# Autodesk Inventor assembly: Manipulator
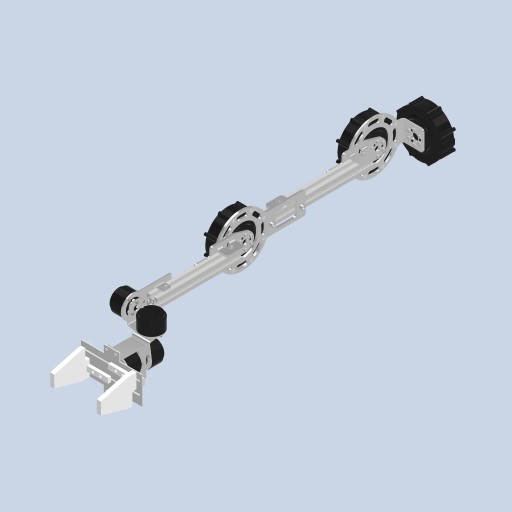
[picture p0: Inventor's stored thumbnail of the model, 512x512]
Saved by Autodesk Inventor 2023 (Build 270158000, 158)
## iProperties
Created: 2024-11-08
Part Number: Manipulator
Document SubType Name: Assembly
Designer: kiyo
Mass: 3708.17 g
Surface Area: 3992.73 cm^2
Volume: 794.407 cm^3
Density: 4.66785 g/cm^3
Author: kiyo
## Documents named in this file (20)
- D:\GitHub\inventor\syu-si\OfficeRobot\Manipulator\Manipulator.iam
- D:\GitHub\inventor\syu-si\OfficeRobot\ReadyMade\Steadywin\GIM8108-8.iam
- D:\GitHub\inventor\syu-si\OfficeRobot\ReadyMade\Steadywin\GIM3505-8_with-driver.ipt
- D:\GitHub\inventor\syu-si\OfficeRobot\Manipulator\wrist-pitch-plate.ipt
- D:\GitHub\inventor\syu-si\OfficeRobot\ReadyMade\Screw\FWSJJ-D5-V2_6-T4_5.ipt
- D:\GitHub\inventor\syu-si\OfficeRobot\ReadyMade\Screw\HNTU5-5.ipt
- D:\GitHub\inventor\syu-si\OfficeRobot\Manipulator\sholder_roll_bracket.ipt
- D:\GitHub\inventor\syu-si\OfficeRobot\ReadyMade\Screw\SCB5-8.ipt
- D:\GitHub\inventor\syu-si\OfficeRobot\ReadyMade\Aluminum-frame\NFS5-2020-170-AV15-BV145.ipt
- D:\GitHub\inventor\syu-si\OfficeRobot\Manipulator\wrist_bracket.ipt
- D:\GitHub\inventor\syu-si\OfficeRobot\Hand\Hand.iam
- D:\GitHub\inventor\syu-si\OfficeRobot\Manipulator\pitch_plate.ipt
- D:\GitHub\inventor\syu-si\OfficeRobot\ReadyMade\Screw\SCB5-25.ipt
- D:\GitHub\inventor\syu-si\OfficeRobot\ReadyMade\Screw\SCB5-10.ipt
- D:\GitHub\inventor\syu-si\OfficeRobot\Manipulator\elbow-pitch-plate_T4.ipt
- D:\GitHub\inventor\syu-si\OfficeRobot\ReadyMade\Screw\HFBCM3-8.ipt
- D:\GitHub\inventor\syu-si\OfficeRobot\ReadyMade\Aluminum-frame\NFS5-2020-215-AV15-BV180.ipt
- D:\GitHub\inventor\syu-si\OfficeRobot\ReadyMade\Screw\CBE3-8.ipt
- D:\GitHub\inventor\syu-si\OfficeRobot\ReadyMade\Screw\CSH-316L-M2_5-6.ipt
- D:\GitHub\inventor\syu-si\OfficeRobot\ReadyMade\Screw\CSH-316L-M2_5-10.ipt
## Components (101 placed, 19 different names)
1. sholder_roll_bracket:1 — 挿入:350, 挿入:414, 挿入:493, 挿入:517, 挿入:526, 挿入:527, 挿入:528, 挿入:529, 挿入:530, 挿入:531, 挿入:532, 挿入:533, 挿入:555, 挿入:556, 挿入:557, 挿入:558, 挿入:559, 挿入:573
2. pitch_plate:1 — 挿入:512, 正接:78, 正接:79, 正接:80, 角度:96, 挿入:561, 挿入:562, 挿入:563, 挿入:564, 挿入:565, 挿入:566
3. elbow-pitch-plate_T4:1 — 挿入:514, 挿入:515, 正接:83, 挿入:518, 挿入:519, 挿入:520, 挿入:521, 挿入:522, 挿入:523, 挿入:524, 挿入:525, 正接:84, 正接:85
4. pitch_plate:2 — 挿入:513, メイト:114, メイト:115, 正接:77, 正接:81, 正接:82, 角度:97, 挿入:567, 挿入:568, 挿入:569, 挿入:570, 挿入:571, 挿入:572, 正接:86
5. wrist-pitch-plate:1 — メイト:71, メイト:72, 正接:48, 正接:49, 角度:76, 角度:77, 角度:78, 正接:50, 正接:51, 挿入:470, 挿入:471
6. wrist_bracket:1
7. wrist_bracket:2 — 挿入:485
8. NFS5-2020-215-AV15-BV180:1
9. NFS5-2020-170-AV15-BV145:1 — メイト:106, メイト:107, 角度:90, 角度:91, 正接:70, 正接:71, 角度:92, メイト:108, 正接:74, 正接:75, メイト:114, メイト:115
10. Hand:1 [sub-assembly] — 挿入:497, 角度:98, 角度:99
11. CSH-316L-M2_5-6:1
12. CSH-316L-M2_5-6:2
13. CSH-316L-M2_5-6:3
14. CSH-316L-M2_5-6:4
15. CSH-316L-M2_5-6:5
16. CSH-316L-M2_5-6:6
17. CSH-316L-M2_5-6:7
18. CSH-316L-M2_5-6:8
19. CSH-316L-M2_5-6:9
20. CSH-316L-M2_5-10:1
21. CSH-316L-M2_5-10:2
22. CSH-316L-M2_5-10:3
23. CSH-316L-M2_5-10:4
24. CSH-316L-M2_5-10:5
25. CSH-316L-M2_5-10:6
26. CSH-316L-M2_5-10:7
27. CSH-316L-M2_5-10:8
28. CSH-316L-M2_5-10:9
29. CBE3-8:1 — 挿入:555
30. CBE3-8:2 — 挿入:557
31. CBE3-8:3 — 挿入:558
32. CBE3-8:4 — 挿入:573
33. CBE3-8:5 — 挿入:556
34. CBE3-8:6 — 挿入:559
35. CBE3-8:7 — 挿入:562
36. CBE3-8:8 — 挿入:561
37. CBE3-8:9 — 挿入:569
38. CBE3-8:10 — 挿入:572
39. CBE3-8:11 — 挿入:568
40. CBE3-8:12 — 挿入:563
41. CBE3-8:13 — 挿入:566
42. CBE3-8:14 — 挿入:567
43. CBE3-8:15 — 挿入:570
44. CBE3-8:16 — 挿入:571
45. CBE3-8:17 — 挿入:565
46. CBE3-8:18 — 挿入:564
47. HFBCM3-8:1 — 挿入:521
48. HFBCM3-8:2 — 挿入:524
49. HFBCM3-8:3 — 挿入:525
50. HFBCM3-8:4 — 挿入:523
51. HFBCM3-8:5 — 挿入:522
52. HFBCM3-8:6 — 挿入:518
53. HFBCM3-8:7 — 挿入:519
54. HFBCM3-8:8 — 挿入:520
55. HFBCM3-8:9 — 挿入:531
56. HFBCM3-8:10 — 挿入:532
57. HFBCM3-8:11 — 挿入:530
58. HFBCM3-8:12 — 挿入:529
59. HFBCM3-8:13 — 挿入:528
60. HFBCM3-8:14 — 挿入:533
61. HFBCM3-8:15 — 挿入:526
62. HFBCM3-8:16 — 挿入:527
63. FWSJJ-D5-V2_6-T4_5:16
64. FWSJJ-D5-V2_6-T4_5:17
65. FWSJJ-D5-V2_6-T4_5:18
66. FWSJJ-D5-V2_6-T4_5:10
67. FWSJJ-D5-V2_6-T4_5:11
68. FWSJJ-D5-V2_6-T4_5:12
69. FWSJJ-D5-V2_6-T4_5:13
70. FWSJJ-D5-V2_6-T4_5:14
71. FWSJJ-D5-V2_6-T4_5:15
72. SCB5-25:1 — 正接:78
73. SCB5-25:2 — メイト:108, 正接:74, 正接:75, 正接:77
74. SCB5-25:3 — 挿入:516, 正接:83
75. SCB5-25:4
76. SCB5-10:1 — 正接:80
77. SCB5-10:2 — 正接:79
78. SCB5-10:3 — メイト:106, 正接:70, 正接:82
79. SCB5-10:4 — メイト:107, 正接:71, 正接:81
80. SCB5-10:5 — 正接:85
81. SCB5-10:6 — 正接:84, 正接:86
82. SCB5-8:1 — 挿入:412, メイト:72, 正接:49, 正接:50
83. SCB5-8:2 — 挿入:411, メイト:71, 正接:48, 正接:51
84. HNTU5-5:1 — 角度:78
85. HNTU5-5:2 — 挿入:412, 角度:76
86. HNTU5-5:3 — 挿入:411, 角度:77
87. HNTU5-5:4 — 挿入:516
88. HNTU5-5:5
89. HNTU5-5:6
90. HNTU5-5:7
91. HNTU5-5:8 — 角度:90
92. HNTU5-5:9 — 角度:91
93. HNTU5-5:10 — 角度:92
94. HNTU5-5:11
95. HNTU5-5:12
96. GIM8108-8:1 [sub-assembly] — 挿入:350, 肩ピッチとの角度関係, 環境固定, 環境固定2
97. GIM8108-8:2 [sub-assembly] — 挿入:414, 肩ピッチとの角度関係, 挿入:493, 挿入:512, 角度:96, 挿入:517
98. GIM8108-8:3 [sub-assembly] — 挿入:513, 挿入:514, 挿入:515, 角度:97
99. GIM3505-8_with-driver:9 — 挿入:470, 挿入:471
100. GIM3505-8_with-driver:8 — 挿入:485
101. GIM3505-8_with-driver:10 — 挿入:497
## Relationships (157: Insert 90, Tangent 26, Mate 23, Angle 18)
- 挿入:350 [Insert]: sholder_roll_bracket:1 ↔ GIM8108-8:1
- [Insert] (-3.2 mm): SCB5-25:4 ↔ HNTU5-5:1
- [Insert]: wrist_bracket:1 ↔ CSH-316L-M2_5-6:1
- [Insert]: wrist_bracket:1 ↔ CSH-316L-M2_5-6:2
- [Insert]: wrist_bracket:1 ↔ CSH-316L-M2_5-6:3
- [Insert]: wrist_bracket:1 ↔ GIM3505-8_with-driver:8
- [Insert]: wrist_bracket:1 ↔ GIM3505-8_with-driver:8
- [Insert]: wrist_bracket:1 ↔ CSH-316L-M2_5-10:1
- [Insert]: wrist_bracket:1 ↔ CSH-316L-M2_5-10:2
- [Insert]: wrist_bracket:1 ↔ CSH-316L-M2_5-10:3
- [Insert]: wrist_bracket:1 ↔ FWSJJ-D5-V2_6-T4_5:11
- [Insert]: wrist_bracket:1 ↔ FWSJJ-D5-V2_6-T4_5:12
- [Insert]: wrist_bracket:1 ↔ FWSJJ-D5-V2_6-T4_5:10
- 挿入:411 [Insert] (3.2 mm): SCB5-8:2 ↔ HNTU5-5:3
- 挿入:412 [Insert] (3.2 mm): SCB5-8:1 ↔ HNTU5-5:2
- 挿入:414 [Insert]: sholder_roll_bracket:1 ↔ GIM8108-8:2
- [Insert] (2 mm): CSH-316L-M2_5-10:4 ↔ FWSJJ-D5-V2_6-T4_5:17
- [Insert] (2 mm): CSH-316L-M2_5-10:5 ↔ FWSJJ-D5-V2_6-T4_5:16
- [Insert] (2 mm): CSH-316L-M2_5-10:6 ↔ FWSJJ-D5-V2_6-T4_5:18
- [Insert]: wrist_bracket:2 ↔ CSH-316L-M2_5-10:4
- [Insert]: wrist_bracket:2 ↔ CSH-316L-M2_5-10:5
- [Insert]: wrist_bracket:2 ↔ CSH-316L-M2_5-10:6
- [Insert]: wrist_bracket:2 ↔ GIM3505-8_with-driver:10
- [Insert]: wrist_bracket:2 ↔ GIM3505-8_with-driver:10
- 肩ピッチとの角度関係 [Angle] (0 deg): GIM8108-8:1 ↔ GIM8108-8:2
- 環境固定 [Angle] (-90 deg): GIM8108-8:1
- [Mate]: wrist-pitch-plate:1 ↔ SCB5-25:4
- メイト:71 [Mate]: wrist-pitch-plate:1 ↔ SCB5-8:2
- メイト:72 [Mate]: wrist-pitch-plate:1 ↔ SCB5-8:1
- [Tangent] (0.25 mm): wrist-pitch-plate:1 ↔ SCB5-25:4
- [Tangent] (7.5 mm): wrist-pitch-plate:1 ↔ SCB5-25:4
- 正接:48 [Tangent] (0.25 mm): wrist-pitch-plate:1 ↔ SCB5-8:2
- 正接:49 [Tangent] (0.25 mm): wrist-pitch-plate:1 ↔ SCB5-8:1
- 角度:76 [Angle] (0 deg): wrist-pitch-plate:1 ↔ HNTU5-5:2
- 角度:77 [Angle] (0 deg): wrist-pitch-plate:1 ↔ HNTU5-5:3
- 角度:78 [Angle] (0 deg): wrist-pitch-plate:1 ↔ HNTU5-5:1
- 正接:50 [Tangent] (7.5 mm): wrist-pitch-plate:1 ↔ SCB5-8:1
- 正接:51 [Tangent] (7.5 mm): wrist-pitch-plate:1 ↔ SCB5-8:2
- 挿入:470 [Insert]: wrist-pitch-plate:1 ↔ GIM3505-8_with-driver:9
- 挿入:471 [Insert]: wrist-pitch-plate:1 ↔ GIM3505-8_with-driver:9
- [Mate] (1 mm): NFS5-2020-215-AV15-BV180:1 ↔ HNTU5-5:4
- [Tangent] (32.5 mm): NFS5-2020-215-AV15-BV180:1 ↔ SCB5-25:3
- [Insert] (5.2 mm): SCB5-10:6 ↔ HNTU5-5:11
- [Angle] (0 deg): NFS5-2020-215-AV15-BV180:1 ↔ HNTU5-5:11
- [Mate] (1 mm): NFS5-2020-215-AV15-BV180:1 ↔ HNTU5-5:11
- [Insert] (5.2 mm): SCB5-10:5 ↔ HNTU5-5:12
- [Mate] (1 mm): NFS5-2020-215-AV15-BV180:1 ↔ HNTU5-5:12
- [Mate]: wrist-pitch-plate:1 ↔ NFS5-2020-170-AV15-BV145:1
- [Mate]: wrist-pitch-plate:1 ↔ NFS5-2020-170-AV15-BV145:1
- [Tangent] (22.5 mm): NFS5-2020-170-AV15-BV145:1 ↔ SCB5-25:4
- 挿入:485 [Insert] (4.5 mm): wrist_bracket:2 ↔ GIM3505-8_with-driver:8
- [Insert] (4.5 mm): wrist_bracket:1 ↔ GIM3505-8_with-driver:9
- 環境固定2 [Angle] (0 deg): GIM8108-8:1
- 挿入:493 [Insert]: sholder_roll_bracket:1 ↔ GIM8108-8:2
- [Insert]: wrist-pitch-plate:1 ↔ CSH-316L-M2_5-6:4
- [Insert]: wrist-pitch-plate:1 ↔ CSH-316L-M2_5-6:6
- [Insert]: wrist-pitch-plate:1 ↔ CSH-316L-M2_5-6:5
- 挿入:497 [Insert] (4.5 mm): Hand:1 ↔ GIM3505-8_with-driver:10
- [Insert] (1.5 mm): CSH-316L-M2_5-10:7 ↔ FWSJJ-D5-V2_6-T4_5:13
- [Insert] (1.5 mm): CSH-316L-M2_5-10:9 ↔ FWSJJ-D5-V2_6-T4_5:15
- [Insert] (1.5 mm): CSH-316L-M2_5-10:8 ↔ FWSJJ-D5-V2_6-T4_5:14
- [Insert]: Hand:1 ↔ CSH-316L-M2_5-10:9
- [Insert]: Hand:1 ↔ CSH-316L-M2_5-10:8
- [Insert]: Hand:1 ↔ CSH-316L-M2_5-10:7
- [Insert] (-2.2 mm): SCB5-25:1 ↔ HNTU5-5:6
- [Tangent] (12.5 mm): NFS5-2020-215-AV15-BV180:1 ↔ SCB5-25:1
- [Angle] (0 deg): NFS5-2020-215-AV15-BV180:1 ↔ HNTU5-5:6
- [Insert] (5.2 mm): SCB5-10:1 ↔ HNTU5-5:7
- [Insert] (5.2 mm): SCB5-10:2 ↔ HNTU5-5:5
- [Tangent] (7.5 mm): NFS5-2020-215-AV15-BV180:1 ↔ SCB5-10:2
- [Tangent] (7.5 mm): NFS5-2020-215-AV15-BV180:1 ↔ SCB5-10:1
- [Insert] (5.2 mm): SCB5-10:3 ↔ HNTU5-5:8
- [Insert] (5.2 mm): SCB5-10:4 ↔ HNTU5-5:9
- メイト:106 [Mate] (4 mm): NFS5-2020-170-AV15-BV145:1 ↔ SCB5-10:3
- メイト:107 [Mate] (4 mm): NFS5-2020-170-AV15-BV145:1 ↔ SCB5-10:4
- 角度:90 [Angle] (0 deg): NFS5-2020-170-AV15-BV145:1 ↔ HNTU5-5:8
- 角度:91 [Angle] (0 deg): NFS5-2020-170-AV15-BV145:1 ↔ HNTU5-5:9
- 正接:70 [Tangent] (7.5 mm): NFS5-2020-170-AV15-BV145:1 ↔ SCB5-10:3
- 正接:71 [Tangent] (7.5 mm): NFS5-2020-170-AV15-BV145:1 ↔ SCB5-10:4
- [Insert] (-2.2 mm): SCB5-25:2 ↔ HNTU5-5:10
- 角度:92 [Angle] (0 deg): NFS5-2020-170-AV15-BV145:1 ↔ HNTU5-5:10
- メイト:108 [Mate] (4 mm): NFS5-2020-170-AV15-BV145:1 ↔ SCB5-25:2
- 正接:74 [Tangent] (12.5 mm): NFS5-2020-170-AV15-BV145:1 ↔ SCB5-25:2
- 正接:75 [Tangent] (7.5 mm): NFS5-2020-170-AV15-BV145:1 ↔ SCB5-25:2
- [Mate] (4 mm): NFS5-2020-215-AV15-BV180:1 ↔ SCB5-25:1
- [Tangent] (7.5 mm): NFS5-2020-215-AV15-BV180:1 ↔ SCB5-25:1
- [Mate] (4 mm): NFS5-2020-215-AV15-BV180:1 ↔ SCB5-10:1
- [Mate] (4 mm): NFS5-2020-215-AV15-BV180:1 ↔ SCB5-10:2
- 挿入:512 [Insert]: pitch_plate:1 ↔ GIM8108-8:2
- 挿入:513 [Insert]: pitch_plate:2 ↔ GIM8108-8:3
- [Mate]: pitch_plate:1 ↔ NFS5-2020-215-AV15-BV180:1
- [Mate]: pitch_plate:1 ↔ NFS5-2020-215-AV15-BV180:1
- メイト:114 [Mate]: pitch_plate:2 ↔ NFS5-2020-170-AV15-BV145:1
- メイト:115 [Mate]: pitch_plate:2 ↔ NFS5-2020-170-AV15-BV145:1
- 正接:77 [Tangent] (0.25 mm): pitch_plate:2 ↔ SCB5-25:2
- 正接:78 [Tangent] (0.25 mm): pitch_plate:1 ↔ SCB5-25:1
- [Angle] (0 deg): NFS5-2020-215-AV15-BV180:1 ↔ HNTU5-5:7
- [Angle] (0 deg): NFS5-2020-215-AV15-BV180:1 ↔ HNTU5-5:5
- 正接:79 [Tangent] (0.25 mm): pitch_plate:1 ↔ SCB5-10:2
- 正接:80 [Tangent] (0.25 mm): pitch_plate:1 ↔ SCB5-10:1
- 正接:81 [Tangent] (0.25 mm): pitch_plate:2 ↔ SCB5-10:4
- 正接:82 [Tangent] (0.25 mm): pitch_plate:2 ↔ SCB5-10:3
- 挿入:514 [Insert]: elbow-pitch-plate_T4:1 ↔ GIM8108-8:3
- 挿入:515 [Insert]: elbow-pitch-plate_T4:1 ↔ GIM8108-8:3
- [Angle] (0 deg): NFS5-2020-215-AV15-BV180:1 ↔ HNTU5-5:4
- 挿入:516 [Insert] (-2.2 mm): SCB5-25:3 ↔ HNTU5-5:4
- [Mate] (4 mm): NFS5-2020-215-AV15-BV180:1 ↔ SCB5-25:3
- [Mate]: NFS5-2020-215-AV15-BV180:1 ↔ HNTU5-5:11
- [Mate]: NFS5-2020-215-AV15-BV180:1 ↔ HNTU5-5:12
- [Mate]: elbow-pitch-plate_T4:1 ↔ NFS5-2020-215-AV15-BV180:1
- [Mate]: elbow-pitch-plate_T4:1 ↔ NFS5-2020-215-AV15-BV180:1
- 正接:83 [Tangent] (0.25 mm): elbow-pitch-plate_T4:1 ↔ SCB5-25:3
- 角度:96 [Angle] (0 deg): pitch_plate:1 ↔ GIM8108-8:2
- 角度:97 [Angle] (0 deg): pitch_plate:2 ↔ GIM8108-8:3
- 角度:98 [Angle] (0 deg): Hand:1
- 角度:99 [Angle] (0 deg): Hand:1
- 挿入:517 [Insert]: sholder_roll_bracket:1 ↔ GIM8108-8:2
- 挿入:518 [Insert]: elbow-pitch-plate_T4:1 ↔ HFBCM3-8:6
- 挿入:519 [Insert]: elbow-pitch-plate_T4:1 ↔ HFBCM3-8:7
- 挿入:520 [Insert]: elbow-pitch-plate_T4:1 ↔ HFBCM3-8:8
- 挿入:521 [Insert]: elbow-pitch-plate_T4:1 ↔ HFBCM3-8:1
- 挿入:522 [Insert]: elbow-pitch-plate_T4:1 ↔ HFBCM3-8:5
- 挿入:523 [Insert]: elbow-pitch-plate_T4:1 ↔ HFBCM3-8:4
- 挿入:524 [Insert]: elbow-pitch-plate_T4:1 ↔ HFBCM3-8:2
- 挿入:525 [Insert]: elbow-pitch-plate_T4:1 ↔ HFBCM3-8:3
- 挿入:526 [Insert]: sholder_roll_bracket:1 ↔ HFBCM3-8:15
- 挿入:527 [Insert]: sholder_roll_bracket:1 ↔ HFBCM3-8:16
- 挿入:528 [Insert]: sholder_roll_bracket:1 ↔ HFBCM3-8:13
- 挿入:529 [Insert]: sholder_roll_bracket:1 ↔ HFBCM3-8:12
- 挿入:530 [Insert]: sholder_roll_bracket:1 ↔ HFBCM3-8:11
- 挿入:531 [Insert]: sholder_roll_bracket:1 ↔ HFBCM3-8:9
- 挿入:532 [Insert]: sholder_roll_bracket:1 ↔ HFBCM3-8:10
- 挿入:533 [Insert]: sholder_roll_bracket:1 ↔ HFBCM3-8:14
- 正接:84 [Tangent] (0.25 mm): elbow-pitch-plate_T4:1 ↔ SCB5-10:6
- 正接:85 [Tangent] (0.25 mm): elbow-pitch-plate_T4:1 ↔ SCB5-10:5
- [Insert]: wrist_bracket:2 ↔ CSH-316L-M2_5-6:7
- [Insert]: wrist_bracket:2 ↔ CSH-316L-M2_5-6:8
- [Insert]: wrist_bracket:2 ↔ CSH-316L-M2_5-6:9
- 挿入:555 [Insert]: sholder_roll_bracket:1 ↔ CBE3-8:1
- 挿入:556 [Insert]: sholder_roll_bracket:1 ↔ CBE3-8:5
- 挿入:557 [Insert]: sholder_roll_bracket:1 ↔ CBE3-8:2
- 挿入:558 [Insert]: sholder_roll_bracket:1 ↔ CBE3-8:3
- 挿入:559 [Insert]: sholder_roll_bracket:1 ↔ CBE3-8:6
- 挿入:561 [Insert]: pitch_plate:1 ↔ CBE3-8:8
- 挿入:562 [Insert]: pitch_plate:1 ↔ CBE3-8:7
- 挿入:563 [Insert]: pitch_plate:1 ↔ CBE3-8:12
- 挿入:564 [Insert]: pitch_plate:1 ↔ CBE3-8:18
- 挿入:565 [Insert]: pitch_plate:1 ↔ CBE3-8:17
- 挿入:566 [Insert]: pitch_plate:1 ↔ CBE3-8:13
- 挿入:567 [Insert]: pitch_plate:2 ↔ CBE3-8:14
- 挿入:568 [Insert]: pitch_plate:2 ↔ CBE3-8:11
- 挿入:569 [Insert]: pitch_plate:2 ↔ CBE3-8:9
- 挿入:570 [Insert]: pitch_plate:2 ↔ CBE3-8:15
- 挿入:571 [Insert]: pitch_plate:2 ↔ CBE3-8:16
- 挿入:572 [Insert]: pitch_plate:2 ↔ CBE3-8:10
- 挿入:573 [Insert]: sholder_roll_bracket:1 ↔ CBE3-8:4
- 正接:86 [Tangent]: pitch_plate:2 ↔ SCB5-10:6
## Named parameters: d516_d512 = 0 mm, d517_d513 = 0 mm, d519_d268 = 0 mm, d520_d269 = 0 mm, d521_d270 = 0 mm, d782_d733_d492_d466 = 5.2 mm, d787_d782_d733_d492_d466 = 5.2 mm, d14_d733_d492_d466 = 5.2 mm, d880_d14_d733_d492_d466 = 5.2 mm, d889_d14_d733_d492_d466 = 5.2 mm, d890_d14_d733_d492_d466 = 5.2 mm, d900_d25 = -2.2 mm
